# Autodesk Inventor assembly: Ensamblaje_completo
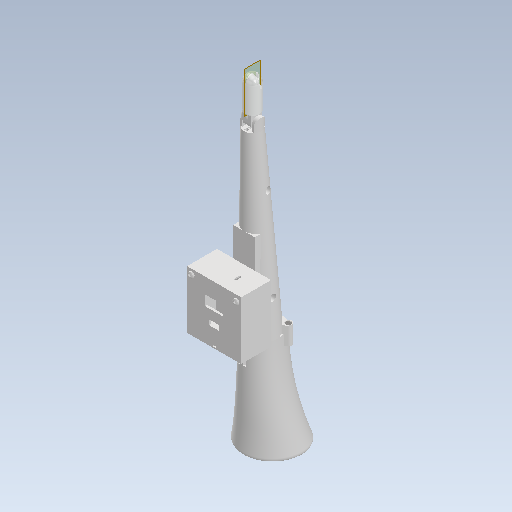
[picture p0: Inventor's stored thumbnail of the model, 512x512]
Saved by Autodesk Inventor 2021 (Build 250183000, 183)
## iProperties
Created: 2023-09-03
Part Number: Ensamblaje_completo
Document SubType Name: Assembly
Designer: Sergio
Author: Sergio
## Documents named in this file (6)
- D:\Sergio\OneDrive - Escuela Superior Politécnica del Litoral\Documentos\12vo Semestre (último)\Diseño Mecatrónico\Proyecto\Diseño Mecánico\solucion GANADORA\Ensamblaje_completo.iam
- D:\Sergio\OneDrive - Escuela Superior Politécnica del Litoral\Documentos\12vo Semestre (último)\Diseño Mecatrónico\Proyecto\Diseño Mecánico\solucion GANADORA\Base\base.iam
- D:\Sergio\OneDrive - Escuela Superior Politécnica del Litoral\Documentos\12vo Semestre (último)\Diseño Mecatrónico\Proyecto\Diseño Mecánico\solucion GANADORA\Caja\Caja.iam
- D:\Sergio\OneDrive - Escuela Superior Politécnica del Litoral\Documentos\12vo Semestre (último)\Diseño Mecatrónico\Proyecto\Diseño Mecánico\solucion GANADORA\dedo\Dedo.iam
- D:\Sergio\OneDrive - Escuela Superior Politécnica del Litoral\Documentos\12vo Semestre (último)\Diseño Mecatrónico\Proyecto\Diseño Mecánico\solucion GANADORA\dedo\Pasador de junta.ipt
- D:\Sergio\Documents\Inventor\Content Center Files\R2021\es-ES\DIN 7985 (H)\DIN 7985 (H) - M4x10-H.ipt
## Components (6 placed, 5 different names)
1. base:1 [sub-assembly] — Coincidencia:1, Tangente:1, Coincidencia:8, Coincidencia:9, Coincidencia:10
2. Caja:1 [sub-assembly] — Coincidencia:4, Coincidencia:5, Coincidencia:6, Coincidencia:7, Coincidencia:10
3. Dedo:1 [sub-assembly] — Coincidencia:1, Coincidencia:2, Coincidencia:3
4. Pasador de junta:1 — Coincidencia:2, Coincidencia:3, Tangente:1
5. DIN 7985 (H) M4x10-H:1 — Coincidencia:4, Coincidencia:5, Coincidencia:8
6. DIN 7985 (H) M4x10-H:2 — Coincidencia:6, Coincidencia:7, Coincidencia:9
## Relationships (11: Mate 10, Tangent 1)
- Coincidencia:1 [Mate]: base:1 ↔ Dedo:1
- Coincidencia:2 [Mate]: Dedo:1 ↔ Pasador de junta:1
- Coincidencia:3 [Mate]: Dedo:1 ↔ Pasador de junta:1
- Tangente:1: base:1 ↔ Pasador de junta:1
- Coincidencia:4 [Mate]: Caja:1 ↔ DIN 7985 (H) M4x10-H:1
- Coincidencia:5 [Mate]: Caja:1 ↔ DIN 7985 (H) M4x10-H:1
- Coincidencia:6 [Mate]: Caja:1 ↔ DIN 7985 (H) M4x10-H:2
- Coincidencia:7 [Mate]: Caja:1 ↔ DIN 7985 (H) M4x10-H:2
- Coincidencia:8 [Mate]: base:1 ↔ DIN 7985 (H) M4x10-H:1
- Coincidencia:9 [Mate]: base:1 ↔ DIN 7985 (H) M4x10-H:2
- Coincidencia:10 [Mate]: base:1 ↔ Caja:1
